# Autodesk Inventor assembly: StartModule
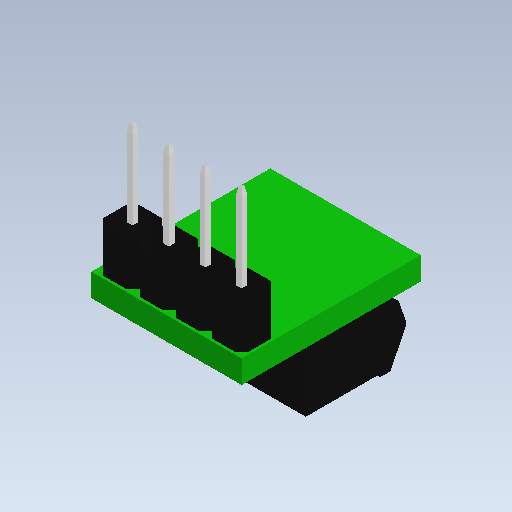
[picture p0: Inventor's stored thumbnail of the model, 512x512]
Saved by Autodesk Inventor 2021 (Build 250183000, 183)
## iProperties
Created: 2021-09-12
Part Number: StartModule
Document SubType Name: Assembly
Designer: ermoz
Author: ermoz
## Documents named in this file (5)
- D:\Moje Wyczyny\My_Poor_Projects\Sneak100_MiniSumo\minisumo-sneak100\mechanics\ElectricElements\StartModule.iam
- D:\Moje Wyczyny\My_Poor_Projects\Sneak100_MiniSumo\minisumo-sneak100\mechanics\ElectricElements\StartModuleBoard.ipt
- D:\Moje Wyczyny\My_Poor_Projects\Sneak100_MiniSumo\minisumo-sneak100\mechanics\ElectricElements\MaleHeaderPin_1x4.iam
- D:\Moje Wyczyny\My_Poor_Projects\Sneak100_MiniSumo\minisumo-sneak100\mechanics\ElectricElements\TSOP4838.ipt
- D:\Moje Wyczyny\My_Poor_Projects\Sneak100_MiniSumo\minisumo-sneak100\mechanics\ElectricElements\Led_0603.ipt
## Components (4 placed, 4 different names)
1. StartModuleBoard:1 — Mate:1, Flush:1, Flush:2, Mate:2, Mate:3
2. MaleHeaderPin_1x4:1 [sub-assembly] — Mate:1, Flush:1, Flush:2
3. TSOP4838:1 — Mate:3
4. Led_0603:1 — Mate:2
## Relationships (5: Mate 3, Flush 2)
- Mate:1: StartModuleBoard:1 ↔ MaleHeaderPin_1x4:1
- Flush:1 (0.17 mm): StartModuleBoard:1 ↔ MaleHeaderPin_1x4:1
- Flush:2 (0.17 mm): StartModuleBoard:1 ↔ MaleHeaderPin_1x4:1
- Mate:2: StartModuleBoard:1 ↔ Led_0603:1
- Mate:3 (1 mm): StartModuleBoard:1 ↔ TSOP4838:1
